# Autodesk Inventor assembly: Gamecube Controller
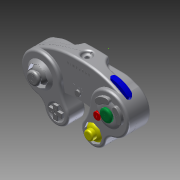
[picture p0: Inventor's stored thumbnail of the model, 180x180]
Saved by Autodesk Inventor 2012 SP1 (Build 160190100, 190)
## iProperties
Created: 2011-12-05
Part Number: Gamecube Controller
Document SubType Name: Assembly
Designer: 133098
Author: 133098
## Documents named in this file (13)
- \\10.1.10.51\2013$\133098\Inventor\Gamecube Controller.iam
- \\10.1.10.51\2013$\133098\Inventor\Top.ipt
- \\10.1.10.51\2013$\133098\Inventor\B Button.ipt
- \\10.1.10.51\2013$\133098\Inventor\Start Button.ipt
- \\10.1.10.51\2013$\133098\Inventor\A Button.ipt
- \\10.1.10.51\2013$\133098\Inventor\D-Pad.ipt
- \\10.1.10.51\2013$\133098\Inventor\X Button.ipt
- \\10.1.10.51\2013$\133098\Inventor\Y Button.ipt
- \\10.1.10.51\2013$\133098\Inventor\Z Button.ipt
- \\10.1.10.51\2013$\133098\Inventor\C Stick.ipt
- \\10.1.10.51\2013$\133098\Inventor\Control Stick.ipt
- \\10.1.10.51\2013$\133098\Inventor\Nintendo.ipt
- \\10.1.10.51\2013$\133098\Inventor\Back.ipt
## Components (12 placed, 12 different names)
1. Top:1 — Mate:1, Mate:4, Flush:1, Mate:5, Mate:6, Mate:7, Mate:8, Mate:9
2. B Button:1 — Mate:1
3. A Button:1
4. D-Pad:1 — Mate:4, Flush:1
5. X Button:1
6. Y Button:1
7. Z Button:1 — Mate:5
8. C Stick:1 — Mate:6
9. Control Stick:1 — Mate:7
10. Start Button:2
11. Nintendo:1 — Mate:8
12. Back:1 — Mate:9
## Relationships (8: Mate 7, Flush 1)
- Mate:1: Top:1 ↔ B Button:1
- Mate:4: Top:1 ↔ D-Pad:1
- Flush:1: Top:1 ↔ D-Pad:1
- Mate:5: Top:1 ↔ Z Button:1
- Mate:6: Top:1 ↔ C Stick:1
- Mate:7: Top:1 ↔ Control Stick:1
- Mate:8: Top:1 ↔ Nintendo:1
- Mate:9: Top:1 ↔ Back:1
